# Autodesk Inventor assembly: 739375
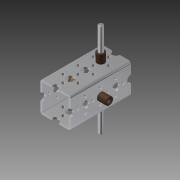
[picture p0: Inventor's stored thumbnail of the model, 180x180]
Saved by Autodesk Inventor 2015 SP1 (Build 190203100, 203)
## iProperties
Category: Add-on Components
Company: Autodesk Inc.
Created: 2014-11-26
Part Number: 739375
Document SubType Name: Assembly
Designer: Tetrix
Catalog Web Link: http://www.tetrixrobotics.com/Gears_and_Sprockets/TETRIX_MAX/TETRIX_Worm_Gear_Box
Vendor: Tetrix
Author: Autodesk Inc.
## Documents named in this file (10)
- D:\Data Folder\FTC 2015\KOP\Tetrix\Tetrix_739375.iam
- D:\Data Folder\FTC 2015\KOP\Tetrix\Tetrix_739375_Shaft.ipt
- D:\Data Folder\FTC 2015\KOP\Tetrix\Tetrix_739375_Bushing.ipt
- D:\Data Folder\FTC 2015\KOP\Tetrix\Tetrix_739375_Channel.ipt
- D:\Data Folder\FTC 2015\KOP\Tetrix\Tetrix_739375_BushingSmall.ipt
- D:\Data Folder\FTC 2015\KOP\Tetrix\Tetrix_739375_Worm.ipt
- D:\Data Folder\FTC 2015\KOP\Tetrix\Tetrix_739375_Screw2.ipt
- D:\Data Folder\FTC 2015\KOP\Tetrix\Tetrix_739375_Screw1.ipt
- D:\Data Folder\FTC 2015\KOP\Tetrix\Tetrix_739375_Gear.ipt
- D:\Data Folder\FTC 2015\KOP\Tetrix\Tetrix_739375_Shaft1.ipt
## Components (13 placed, 9 different names)
1. Tetrix_739375_Shaft:1 — Mate:1, Angle:1, Flush:1, Mate:2
2. Tetrix_739375_Bushing:1 — Insert:6, Mate:3
3. Tetrix_739375_Bushing:2 — Insert:4
4. Tetrix_739375_Bushing:3 — Insert:3
5. Tetrix_739375_Channel:1 — Mate:1, Angle:1, Flush:1, Insert:3, Insert:4, Insert:5, Insert:6, Mate:4, Flush:3
6. Tetrix_739375_BushingSmall:1 — Insert:5
7. Tetrix_739375_Worm:1 — Mate:2, Angle:2, Mate:8, Mate:9, Mate:10
8. Tetrix_739375_Screw2:1 — Mate:6, Flush:2
9. Tetrix_739375_Screw2:2 — Mate:5, Flush:2, Symmetry:1
10. Tetrix_739375_Screw1:1 — Mate:9
11. Tetrix_739375_Screw1:2 — Mate:10
12. Tetrix_739375_Gear:1 — Mate:3, Mate:4, Insert:7, Mate:5, Mate:6, Flush:3, Mate:7, Mate:8, Symmetry:1
13. Tetrix_739375_Shaft1:1 — Insert:7
## Relationships (21: Mate 10, Insert 5, Flush 3, Angle 2, Symmetry 1)
- Mate:1: Tetrix_739375_Shaft:1 ↔ Tetrix_739375_Channel:1
- Angle:1 (0 deg): Tetrix_739375_Shaft:1 ↔ Tetrix_739375_Channel:1
- Flush:1 (-34 mm): Tetrix_739375_Shaft:1 ↔ Tetrix_739375_Channel:1
- Insert:3: Tetrix_739375_Bushing:3 ↔ Tetrix_739375_Channel:1
- Mate:2: Tetrix_739375_Shaft:1 ↔ Tetrix_739375_Worm:1
- Insert:4: Tetrix_739375_Bushing:2 ↔ Tetrix_739375_Channel:1
- Insert:5: Tetrix_739375_Channel:1 ↔ Tetrix_739375_BushingSmall:1
- Insert:6: Tetrix_739375_Bushing:1 ↔ Tetrix_739375_Channel:1
- Mate:3: Tetrix_739375_Bushing:1 ↔ Tetrix_739375_Gear:1
- Mate:4: Tetrix_739375_Channel:1 ↔ Tetrix_739375_Gear:1
- Insert:7: Tetrix_739375_Gear:1 ↔ Tetrix_739375_Shaft1:1
- Mate:5: Tetrix_739375_Screw2:2 ↔ Tetrix_739375_Gear:1
- Mate:6: Tetrix_739375_Screw2:1 ↔ Tetrix_739375_Gear:1
- Flush:2: Tetrix_739375_Screw2:1 ↔ Tetrix_739375_Screw2:2
- Flush:3: Tetrix_739375_Channel:1 ↔ Tetrix_739375_Gear:1
- Mate:7: Tetrix_739375_Gear:1
- Angle:2 (90 deg): Tetrix_739375_Worm:1
- Mate:8: Tetrix_739375_Worm:1 ↔ Tetrix_739375_Gear:1
- Symmetry:1: Tetrix_739375_Screw2:2 ↔ Tetrix_739375_Gear:1
- Mate:9: Tetrix_739375_Worm:1 ↔ Tetrix_739375_Screw1:1
- Mate:10: Tetrix_739375_Worm:1 ↔ Tetrix_739375_Screw1:2
